# Autodesk Inventor assembly: splashBase
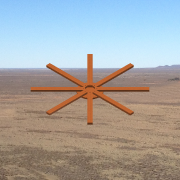
[picture p0: Inventor's stored thumbnail of the model, 180x180]
Saved by Autodesk Inventor 2014 SP1 (Build 180222100, 222)
## iProperties
Created: 2014-05-01
Part Number: splashBase
Document SubType Name: Assembly
Designer: Dave
Author: Dave
## Documents named in this file (3)
- C:\Users\Dave\Desktop\hera-cad\surface\splashBase.iam
- C:\Users\Dave\Desktop\hera-cad\surface\splashBaseDisc.ipt
- C:\Users\Dave\Desktop\hera-cad\surface\splashFurring.ipt
## Components (9 placed, 2 different names)
1. splashBaseDisc:1 — Insert:1
2. splashFurring:1 — Insert:1
3. splashFurring:2
4. splashFurring:3
5. splashFurring:4
6. splashFurring:5
7. splashFurring:6
8. splashFurring:7
9. splashFurring:8
## Component patterns: (8 elements, first: splashFurring:1)
## Relationships (1: Insert 1)
- Insert:1: splashBaseDisc:1 ↔ splashFurring:1
